# Autodesk Inventor assembly: FrontLink
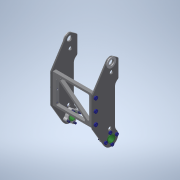
[picture p0: Inventor's stored thumbnail of the model, 180x180]
Saved by Autodesk Inventor 2020.4 (Build 244396000, 396)
## iProperties
Created: 2016-08-23
Part Number: FrontLink
Material: 一般
Document SubType Name: Assembly
Designer: hiro
Mass: 33.5175 g
Surface Area: 182.778 cm^2
Volume: 15.549 cm^3
Density: 2.15561 g/cm^3
Author: hiro
## Documents named in this file (14)
- C:\Users\Masato\Documents\Inventor\CIT Brains_Inventor\OpenPlatform_ver3_0 - ve4_1 branch\LowerBody\Link\FrontLink.iam
- C:\Users\Masato\Documents\Inventor\CIT Brains_Inventor\OpenPlatform_ver3_0 - ve4_1 branch\LowerBody\Link\FrontLink_diagonal.ipt
- C:\Users\Masato\Documents\Inventor\CIT Brains_Inventor\OpenPlatform_ver3_0 - ve4_1 branch\Ready_Made\Screw\M3-6.ipt
- C:\Users\Masato\Documents\Inventor\CIT Brains_Inventor\OpenPlatform_ver3_0 - ve4_1 branch\LowerBody\Link\FrontLink_frame.ipt
- C:\Users\Masato\Documents\Inventor\CIT Brains_Inventor\OpenPlatform_ver3_0 - ve4_1 branch\Ready_Made\Screw\M2_6-10.ipt
- C:\Users\Masato\Documents\Inventor\CIT Brains_Inventor\OpenPlatform_ver3_0 - ve4_1 branch\LowerBody\Knee\Knee_clamp.ipt
- C:\Users\Masato\Documents\Inventor\CIT Brains_Inventor\OpenPlatform_ver3_0 - ve4_1 branch\Ready_Made\WSSS-12-10-8.ipt
- C:\Users\Masato\Documents\Inventor\CIT Brains_Inventor\OpenPlatform_ver3_0 - ve4_1 branch\Ready_Made\TT-0814-10.ipt
- C:\Users\Masato\Documents\Inventor\CIT Brains_Inventor\OpenPlatform_ver3_0 - ve4_1 branch\LowerBody\Link\FrontLink\AIP\FEA\dtq5hwjwg.fins
- C:\Users\Masato\Documents\Inventor\CIT Brains_Inventor\OpenPlatform_ver3_0 - ve4_1 branch\LowerBody\Link\FrontLink\AIP\FEA\dtq5hwjxc.fsat
- C:\Users\Masato\Documents\Inventor\CIT Brains_Inventor\OpenPlatform_ver3_0 - ve4_1 branch\LowerBody\Link\FrontLink\AIP\FEA\dtq5hwjxc.ftes
- C:\Users\Masato\Documents\Inventor\CIT Brains_Inventor\OpenPlatform_ver3_0 - ve4_1 branch\LowerBody\Link\FrontLink\AIP\FEA\dtq5hwjxc.fwiz
- C:\Users\Masato\Documents\Inventor\CIT Brains_Inventor\OpenPlatform_ver3_0 - ve4_1 branch\LowerBody\Link\FrontLink\AIP\FEA\dtq5hwk0w.fmsh
- C:\Users\Masato\Documents\Inventor\CIT Brains_Inventor\OpenPlatform_ver3_0 - ve4_1 branch\LowerBody\Link\FrontLink\AIP\FEA\dtq5hwk0x.fres
## Components (23 placed, 7 different names)
1. FrontLink_diagonal:1 — 挿入:1, 挿入:2, 挿入:3, 挿入:4, 挿入:5, 挿入:6, フラッシュ:1, メイト:1, メイト:2
2. FrontLink_frame:1 — 挿入:1, 挿入:2, 挿入:3, 挿入:7, 挿入:8, 挿入:9, 挿入:25, 挿入:27, 挿入:26, 挿入:28, 挿入:17, 挿入:18, 挿入:19, 挿入:20, 挿入:60
3. FrontLink_frame:2 — 挿入:4, 挿入:5, 挿入:6, 挿入:10, 挿入:11, 挿入:12, 挿入:21, 挿入:22, 挿入:23, 挿入:24, 挿入:31, 挿入:29, 挿入:32, 挿入:30, 挿入:61
4. M3-6:1 — 挿入:7
5. M3-6:2 — 挿入:8
6. M3-6:3 — 挿入:9
7. M3-6:4 — 挿入:10
8. M3-6:5 — 挿入:11
9. M3-6:6 — 挿入:12
10. M2_6-10:1 — 挿入:25
11. M2_6-10:2 — 挿入:26
12. M2_6-10:3 — 挿入:27
13. M2_6-10:4 — 挿入:28
14. M2_6-10:5 — 挿入:29
15. M2_6-10:6 — 挿入:30
16. M2_6-10:7 — 挿入:31
17. M2_6-10:8 — 挿入:32
18. Knee_clamp:1 — 挿入:15, 挿入:17, 挿入:18, 挿入:19, 挿入:20
19. Knee_clamp:2 — 挿入:16, 挿入:21, 挿入:22, 挿入:23, 挿入:24
20. WSSS-12-10-8:1 — 挿入:15
21. WSSS-12-10-8:2 — 挿入:16
22. TT-0814-10:1 — 挿入:60
23. TT-0814-10:2 — 挿入:61
## Relationships (35: Insert 32, Mate 2, Flush 1)
- 挿入:1 [Insert]: FrontLink_diagonal:1 ↔ FrontLink_frame:1
- 挿入:2 [Insert]: FrontLink_diagonal:1 ↔ FrontLink_frame:1
- 挿入:3 [Insert]: FrontLink_diagonal:1 ↔ FrontLink_frame:1
- 挿入:7 [Insert]: FrontLink_frame:1 ↔ M3-6:1
- 挿入:8 [Insert]: FrontLink_frame:1 ↔ M3-6:2
- 挿入:9 [Insert]: FrontLink_frame:1 ↔ M3-6:3
- 挿入:4 [Insert]: FrontLink_diagonal:1 ↔ FrontLink_frame:2
- 挿入:5 [Insert]: FrontLink_diagonal:1 ↔ FrontLink_frame:2
- 挿入:6 [Insert]: FrontLink_diagonal:1 ↔ FrontLink_frame:2
- 挿入:10 [Insert]: FrontLink_frame:2 ↔ M3-6:4
- 挿入:11 [Insert]: FrontLink_frame:2 ↔ M3-6:5
- 挿入:12 [Insert]: FrontLink_frame:2 ↔ M3-6:6
- 挿入:15 [Insert]: Knee_clamp:1 ↔ WSSS-12-10-8:1
- 挿入:16 [Insert]: Knee_clamp:2 ↔ WSSS-12-10-8:2
- 挿入:17 [Insert]: FrontLink_frame:1 ↔ Knee_clamp:1
- 挿入:18 [Insert]: FrontLink_frame:1 ↔ Knee_clamp:1
- 挿入:19 [Insert]: FrontLink_frame:1 ↔ Knee_clamp:1
- 挿入:20 [Insert]: FrontLink_frame:1 ↔ Knee_clamp:1
- 挿入:21 [Insert]: FrontLink_frame:2 ↔ Knee_clamp:2
- 挿入:22 [Insert]: FrontLink_frame:2 ↔ Knee_clamp:2
- 挿入:23 [Insert]: FrontLink_frame:2 ↔ Knee_clamp:2
- 挿入:24 [Insert]: FrontLink_frame:2 ↔ Knee_clamp:2
- 挿入:31 [Insert]: FrontLink_frame:2 ↔ M2_6-10:7
- 挿入:29 [Insert]: FrontLink_frame:2 ↔ M2_6-10:5
- 挿入:32 [Insert]: FrontLink_frame:2 ↔ M2_6-10:8
- 挿入:30 [Insert]: FrontLink_frame:2 ↔ M2_6-10:6
- 挿入:25 [Insert]: FrontLink_frame:1 ↔ M2_6-10:1
- 挿入:27 [Insert]: FrontLink_frame:1 ↔ M2_6-10:3
- 挿入:26 [Insert]: FrontLink_frame:1 ↔ M2_6-10:2
- 挿入:28 [Insert]: FrontLink_frame:1 ↔ M2_6-10:4
- フラッシュ:1 [Flush]: FrontLink_diagonal:1
- メイト:1 [Mate]: FrontLink_diagonal:1
- メイト:2 [Mate]: FrontLink_diagonal:1
- 挿入:60 [Insert]: FrontLink_frame:1 ↔ TT-0814-10:1
- 挿入:61 [Insert]: FrontLink_frame:2 ↔ TT-0814-10:2
## Named parameters: sa_0 = 100000, sa_1 = 100000
note: some values were not read from the file. Shown as the stored number, unit unknown: "sa_0", "sa_1".
